# Autodesk Inventor assembly: Assembly
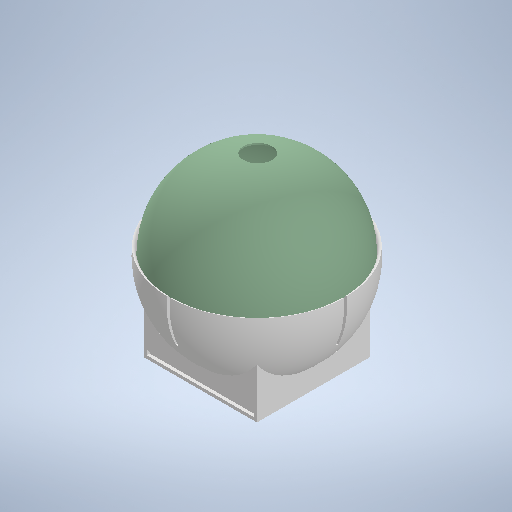
[picture p0: Inventor's stored thumbnail of the model, 512x512]
Saved by Autodesk Inventor 2025 (Build 290162000, 162)
## iProperties
Created: 2024-11-17
Part Number: Assembly
Document SubType Name: Assembly
Designer: ethan
Author: ethan
## Documents named in this file (3)
- C:\Users\ethan\Documents\GitHub\3D-Pants\CameraBall\Assembly.iam
- C:\Users\ethan\Documents\GitHub\3D-Pants\CameraBall\Ball.ipt
- C:\Users\ethan\Documents\GitHub\3D-Pants\CameraBall\Socket.ipt
## Components (2 placed, 2 different names)
1. Ball:1 — Mate:1
2. Socket:1 — Mate:1
## Relationships (1: Mate 1)
- Mate:1: Ball:1 ↔ Socket:1
